# Autodesk Inventor assembly: ASY NDM-VOS_powder_hopper
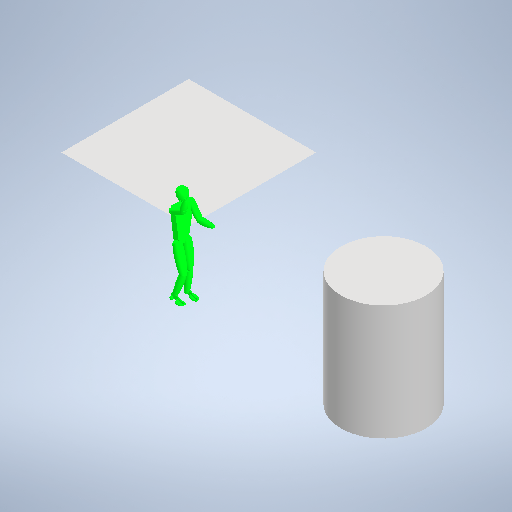
[picture p0: Inventor's stored thumbnail of the model, 512x512]
Saved by Autodesk Inventor 2025 (Build 290162010, 162A)
## iProperties
Created: 2024-07-24
Part Number: ASY NDM-VOS_powder_hopper
Document SubType Name: Assembly
Designer: admin
Author: admin
## Documents named in this file (5)
- C:\Users\user\YandexDisk\домашниий пк\Inventor\NDM-VOS_powder_hopper\ASY NDM-VOS_powder_hopper.iam
- C:\Users\user\YandexDisk\домашниий пк\Inventor\NDM-VOS_powder_hopper\NDM-VOS dummy1.ipt
- C:\Users\user\YandexDisk\домашниий пк\Inventor\NDM-VOS_powder_hopper\Dummy 3.ipt
- C:\Users\user\YandexDisk\домашниий пк\Inventor\NDM-VOS_powder_hopper\NDM-VOS dummy2.ipt
- C:\Users\user\YandexDisk\домашниий пк\Inventor\NDM-VOS_powder_hopper\human 01\ч ASY human dummy 01.iam
## Components (4 placed, 4 different names)
1. NDM-VOS dummy1:1 — Mate:1
2. Dummy 3:1 — Flush:1
3. NDM-VOS dummy2:1 — Mate:1
4. ч ASY human dummy 01:1 [sub-assembly]
## Relationships (2: Flush 1, Mate 1)
- Flush:1: Dummy 3:1
- Mate:1 (-2500 mm): NDM-VOS dummy1:1 ↔ NDM-VOS dummy2:1
